# Autodesk Inventor assembly: CIM Motor Dewalt Shifter 1764
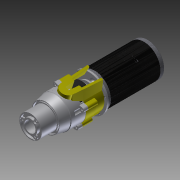
[picture p0: Inventor's stored thumbnail of the model, 180x180]
Saved by Autodesk Inventor 2011 (Build 150239000, 239)
## iProperties
Created: 2008-11-24
Part Number: CIM Motor Dewalt Shifter 1764
Document SubType Name: Assembly
Designer: lwoods
Author: lwoods
## Documents named in this file (11)
- R:\CAD Archives\Motors\CIM Motor Dewalt Shifter 1764\CIM Motor Dewalt Shifter 1764.iam
- R:\CAD Archives\Motors\CIM Motor Dewalt Shifter 1764\CIM Motor 1764.ipt
- R:\CAD Archives\Motors\CIM Motor Dewalt Shifter 1764\Chiaphua Plate 1764.ipt
- R:\CAD Archives\Motors\CIM Motor Dewalt Shifter 1764\Transmission Gear 1764.ipt
- R:\CAD Archives\Motors\CIM Motor Dewalt Shifter 1764\Transmission Top-Hat 1764.ipt
- R:\CAD Archives\Motors\CIM Motor Dewalt Shifter 1764\Switch 1764.ipt
- R:\CAD Archives\Motors\CIM Motor Dewalt Shifter 1764\Cut Drill Handle 1764.ipt
- R:\CAD Archives\Motors\CIM Motor Dewalt Shifter 1764\Cut Drill Handle Mirror 1764.ipt
- R:\CAD Archives\Motors\CIM Motor Dewalt Shifter 1764\Housing 1764.ipt
- R:\CAD Archives\Motors\CIM Motor Dewalt Shifter 1764\Mounting Cover 1764.ipt
- R:\CAD Archives\Motors\CIM Motor Dewalt Shifter 1764\Front Mounting Cover 1764.ipt
## Components (10 placed, 10 different names)
1. CIM Motor 1764:1 — Mate:2, Mate:3, Mate:27, Mate:28
2. Chiaphua Plate 1764:1 — Mate:2, Mate:3, Mate:17, Mate:18, Mate:19, Mate:27, Mate:29
3. Transmission Gear 1764:1 — Mate:4, Mate:5, Mate:6, Mate:14
4. Transmission Top-Hat 1764:1 — Mate:4, Mate:5, Mate:6, Mate:28, Mate:29
5. Cut Drill Handle 1764:1 — Flush:2, Mate:15, Mate:16, Mate:18, Mate:19, Mate:21, Angle:1, Mate:25
6. Cut Drill Handle Mirror 1764:1 — Flush:2, Mate:15, Mate:16, Mate:17, Mate:20
7. Housing 1764:1 — Mate:20, Mate:21, Angle:1, Mate:22, Mate:23, Mate:26
8. Mounting Cover 1764:1 — Mate:24, Angle:2, Flush:3
9. Front Mounting Cover 1764:1 — Mate:22, Mate:23, Mate:24, Angle:2, Flush:3
10. Switch 1764:1 — Mate:25, Mate:26
## Relationships (26: Mate 22, Flush 2, Angle 2)
- Mate:2: CIM Motor 1764:1 ↔ Chiaphua Plate 1764:1
- Mate:3: CIM Motor 1764:1 ↔ Chiaphua Plate 1764:1
- Mate:4: Transmission Gear 1764:1 ↔ Transmission Top-Hat 1764:1
- Mate:5: Transmission Gear 1764:1 ↔ Transmission Top-Hat 1764:1
- Mate:6: Transmission Gear 1764:1 ↔ Transmission Top-Hat 1764:1
- Mate:13
- Mate:14: Transmission Gear 1764:1
- Flush:2: Cut Drill Handle 1764:1 ↔ Cut Drill Handle Mirror 1764:1
- Mate:15: Cut Drill Handle 1764:1 ↔ Cut Drill Handle Mirror 1764:1
- Mate:16: Cut Drill Handle 1764:1 ↔ Cut Drill Handle Mirror 1764:1
- Mate:17: Chiaphua Plate 1764:1 ↔ Cut Drill Handle Mirror 1764:1
- Mate:18: Chiaphua Plate 1764:1 ↔ Cut Drill Handle 1764:1
- Mate:19: Chiaphua Plate 1764:1 ↔ Cut Drill Handle 1764:1
- Mate:20: Cut Drill Handle Mirror 1764:1 ↔ Housing 1764:1
- Mate:21: Cut Drill Handle 1764:1 ↔ Housing 1764:1
- Angle:1 (0 deg): Cut Drill Handle 1764:1 ↔ Housing 1764:1
- Mate:22: Housing 1764:1 ↔ Front Mounting Cover 1764:1
- Mate:23: Housing 1764:1 ↔ Front Mounting Cover 1764:1
- Mate:24: Mounting Cover 1764:1 ↔ Front Mounting Cover 1764:1
- Angle:2 (0 deg): Mounting Cover 1764:1 ↔ Front Mounting Cover 1764:1
- Flush:3: Mounting Cover 1764:1 ↔ Front Mounting Cover 1764:1
- Mate:25: Cut Drill Handle 1764:1 ↔ Switch 1764:1
- Mate:26: Housing 1764:1 ↔ Switch 1764:1
- Mate:27: CIM Motor 1764:1 ↔ Chiaphua Plate 1764:1
- Mate:28: CIM Motor 1764:1 ↔ Transmission Top-Hat 1764:1
- Mate:29: Chiaphua Plate 1764:1 ↔ Transmission Top-Hat 1764:1
